# Autodesk Inventor assembly: body
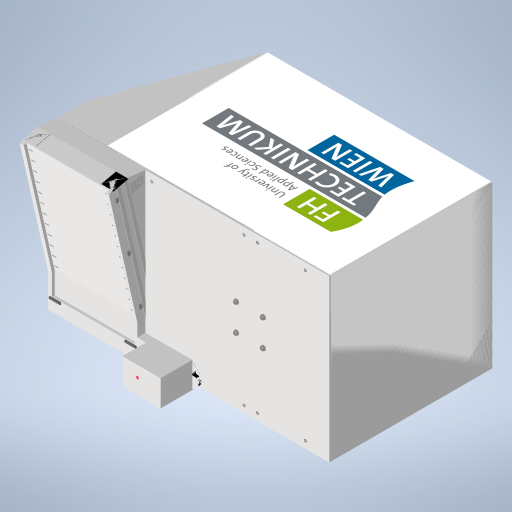
[picture p0: Inventor's stored thumbnail of the model, 512x512]
Saved by Autodesk Inventor 2023 (Build 270158000, 158)
## iProperties
Created: 2023-08-22
Part Number: body
Document SubType Name: Assembly
Designer: chriboehm
Mass: 21023.1 g
Surface Area: 80290.1 cm^2
Volume: 12132.8 cm^3
Density: 1.73275 g/cm^3
Author: chriboehm
## Documents named in this file (28)
- C:\work\robots\butler_2.0\body_model\body.iam
- C:\work\robots\butler_2.0\body_model\parts\Profil 40 x 40 L 450.ipt
- C:\work\robots\butler_2.0\body_model\parts\Profil 40 x 40 L 120.ipt
- C:\work\robots\butler_2.0\body_model\parts\Profil 40 x 40 L 670.ipt
- C:\work\robots\butler_2.0\body_model\parts\Profil 40 x 40 L 540.ipt
- C:\work\robots\butler_2.0\body_model\parts\Profil 40 x 40 L 456.ipt
- C:\work\robots\butler_2.0\body_model\parts\Profil 40 x 40 L 161.ipt
- C:\work\robots\butler_2.0\body_model\parts\Elbow joint 40\Elbow joint 40.iam
- C:\work\robots\butler_2.0\body_model\parts\Reader\RF622A.iam
- C:\work\robots\butler_2.0\body_model\parts\Roller track L 250\Roller track L 250.iam
- C:\work\robots\butler_2.0\body_model\parts\Roller track L 178\Roller track L 178.iam
- C:\work\robots\butler_2.0\body_model\parts\Cap 40_40\Cap 40_40.iam
- C:\work\robots\butler_2.0\body_model\parts\Cap 40_80\Cap 40_80.iam
- C:\work\robots\butler_2.0\body_model\parts\Corner bracket 40_50\Corner bracket 40_50.iam
- C:\work\robots\butler_2.0\body_model\parts\plate_top_01.ipt
- C:\Users\chriboehm\Documents\Inventor\Content Center Files\R2023\en-US\DIN 7984\DIN 7984 - M6 x 12.ipt
- C:\Users\chriboehm\Documents\Inventor\Content Center Files\R2023\en-US\DIN 125-2  A\DIN 125-2 - A 6,4A.ipt
- C:\work\robots\butler_2.0\body_model\parts\plate_top_02.ipt
- C:\work\robots\butler_2.0\body_model\parts\plate_top_03.ipt
- C:\work\robots\butler_2.0\body_model\parts\plate_front.ipt
- C:\work\robots\butler_2.0\body_model\parts\plate_back.ipt
- C:\work\robots\butler_2.0\body_model\parts\plate_side_blank.ipt
- C:\work\robots\butler_2.0\body_model\parts\plate_side_with_logo.ipt
- C:\work\robots\butler_2.0\body_model\parts\emergancy_stop\G_IC03_XX_12648V.iam
- C:\Users\chriboehm\Documents\Inventor\Content Center Files\R2023\en-US\DIN 6912\DIN 6912 - M8 x 20.ipt
- C:\Users\chriboehm\Documents\Inventor\Content Center Files\R2023\en-US\DIN 125-2  A\DIN 125-2 - A 8,4A.ipt
- C:\work\robots\butler_2.0\body_model\body_collision.ipt
- C:\work\robots\butler_2.0\body_model\parts\logo.png
## Components (73 placed, 26 different names)
1. Profil 40 x 40 L 450:1 — Mate:28, Flush:49, Flush:50, Flush:52, Mate:30, Mate:31, Mate:38, Flush:65, Mate:39, Flush:67, Mate:42, Flush:68, Flush:77
2. Profil 40 x 40 L 450:2 — Mate:24, Flush:43, Flush:44, Mate:26, Flush:47, Mate:31, Mate:40, Flush:66, Mate:41, Mate:43, Flush:69, Flush:70, Flush:75
3. Profil 40 x 40 L 120:1 — Mate:33, Flush:55, Flush:56, Mate:34, Flush:57, Flush:58, Angle:2, Angle:3
4. Profil 40 x 40 L 670:1 — Mate:1, Flush:1, Flush:2, Mate:2, Flush:3, Flush:4
5. Profil 40 x 40 L 670:2 — Mate:13, Mate:14, Flush:25, Flush:26, Flush:27, Flush:28, Mate:18, Flush:33, Mate:20, Flush:35, Mate:29, Flush:51, Flush:80, Flush:81, Tangent:2
6. Profil 40 x 40 L 670:3 — Mate:15, Mate:16, Flush:29, Flush:30, Flush:31, Flush:32, Mate:17, Flush:34, Mate:19, Flush:36, Mate:27, Flush:48, Mate:48, Flush:78
7. Profil 40 x 40 L 670:4 — Mate:7, Mate:8, Flush:13, Flush:14, Flush:15, Flush:16
8. Profil 40 x 40 L 540:1 — Mate:5, Flush:9, Flush:10, Mate:8, Flush:13, Flush:14, Mate:10, Flush:17, Flush:18, Mate:13, Flush:27, Flush:28, Mate:22, Flush:39, Flush:40, Flush:79, Mate:99, Mate:104, Mate:113
9. Profil 40 x 40 L 540:2 — Mate:6, Flush:11, Flush:12, Mate:7, Flush:15, Flush:16, Mate:12, Flush:21, Flush:22, Mate:14, Flush:25, Flush:26
10. Profil 40 x 40 L 540:3 — Mate:2, Flush:3, Flush:4, Mate:4, Flush:7, Flush:8, Mate:9, Flush:19, Flush:20, Flush:29, Mate:21, Flush:37, Flush:38
11. Profil 40 x 40 L 540:4 — Mate:1, Flush:1, Flush:2, Mate:3, Flush:5, Flush:6, Mate:11, Flush:23, Flush:24, Mate:15, Flush:31, Mate:97, Flush:85, Mate:101
12. Profil 40 x 40 L 456:1 — Mate:3, Flush:5, Flush:6, Mate:6, Flush:11, Flush:12
13. Profil 40 x 40 L 456:2 — Mate:4, Flush:7, Flush:8, Mate:5, Flush:9, Flush:10
14. Profil 40 x 40 L 456:3 — Mate:11, Mate:12, Flush:21, Flush:22, Flush:23, Flush:24, Flush:32, Mate:46, Mate:78, Flush:82
15. Profil 40 x 40 L 456:4 — Mate:9, Mate:10, Flush:17, Flush:18, Flush:19, Flush:20, Mate:16, Flush:30, Mate:50
16. Profil 40 x 40 L 456:5 — Mate:19, Mate:20, Flush:35, Flush:36, Mate:47, Mate:60
17. Profil 40 x 40 L 456:6 — Mate:17, Mate:18, Flush:33, Flush:34, Mate:46, Mate:47, Tangent:1
18. Profil 40 x 40 L 161:1 — Mate:22, Flush:39, Flush:40, Mate:25, Flush:45, Flush:46, Mate:32, Flush:53, Flush:54, Angle:2, Mate:44, Flush:71, Flush:72
19. Profil 40 x 40 L 161:2 — Mate:21, Flush:37, Flush:38, Mate:23, Flush:41, Flush:42, Mate:45, Flush:73, Flush:74, Mate:49, Flush:76
20. Elbow joint 40:1 [sub-assembly] — Mate:25, Flush:45, Flush:46, Mate:26, Flush:47
21. Elbow joint 40:2 [sub-assembly] — Mate:23, Flush:41, Flush:42, Mate:24, Flush:43, Flush:44
22. Elbow joint 40:3 [sub-assembly] — Mate:27, Flush:48, Mate:28, Flush:49, Flush:50
23. Elbow joint 40:4 [sub-assembly] — Mate:29, Flush:51, Flush:52, Mate:30, Mate:51, Mate:61
24. Elbow joint 40:5 [sub-assembly] — Mate:32, Flush:53, Flush:54, Mate:33, Flush:55, Flush:56
25. Elbow joint 40:6 [sub-assembly] — Mate:34, Flush:57, Flush:58, Mate:95, Flush:83, Flush:84
26. RF622A:1 [sub-assembly] — Mate:95, Flush:83, Flush:84, Angle:3
27. Roller track L 250:1 [sub-assembly] — Mate:37, Flush:63, Flush:64, Mate:40, Flush:66, Mate:41
28. Roller track L 250:2 [sub-assembly] — Flush:61, Flush:62, Mate:36, Mate:38
29. Roller track L 178:1 [sub-assembly] — Mate:37, Flush:63, Flush:64
30. Roller track L 178:2 [sub-assembly] — Flush:61, Flush:62, Mate:36, Flush:65, Mate:39
31. Cap 40_40:1 [sub-assembly] — Mate:45, Flush:73, Flush:74
32. Cap 40_40:4 [sub-assembly] — Mate:44, Flush:71, Flush:72
33. Cap 40_80:1 [sub-assembly] — Mate:43, Flush:69, Flush:70
34. Cap 40_80:2 [sub-assembly] — Flush:67, Mate:42, Flush:68
35. Corner bracket 40_50:1 [sub-assembly] — Mate:48, Flush:77, Flush:78
36. Corner bracket 40_50:2 [sub-assembly] — Mate:49, Flush:75, Flush:76
37. plate_top_01:1 — Mate:50, Flush:79, Mate:51, Mate:56, Mate:57, Mate:58, Mate:59, Mate:100
38. DIN 7984 M6 x 12:1 — Mate:52, Mate:53, Mate:56
39. DIN 7984 M6 x 12:2 — Mate:54, Mate:55, Mate:57
40. DIN 125-2 A A 6,4:1 — Mate:52, Mate:53, Mate:59
41. DIN 125-2 A A 6,4:2 — Mate:54, Mate:55, Mate:58
42. plate_top_02:1 — Mate:60, Mate:61, Flush:80, Mate:70, Mate:71, Mate:72, Mate:73, Mate:74, Mate:75, Mate:76, Mate:102, Mate:105, Mate:107, Mate:108
43. DIN 7984 M6 x 12:3 — Mate:72
44. DIN 125-2 A A 6,4:3 — Mate:73
45. DIN 7984 M6 x 12:4 — Mate:70
46. DIN 125-2 A A 6,4:4 — Mate:71
47. DIN 7984 M6 x 12:5 — Mate:76
48. DIN 125-2 A A 6,4:5 — Mate:109
49. DIN 7984 M6 x 12:6 — Mate:74
50. DIN 125-2 A A 6,4:6 — Mate:75
51. plate_top_03:1 — Mate:78, Flush:81, Flush:82, Mate:87, Mate:88, Mate:89, Mate:90, Mate:91, Mate:92, Mate:93, Mate:94, Mate:98, Mate:122, Mate:123, Mate:124
52. DIN 7984 M6 x 12:7 — Mate:91
53. DIN 125-2 A A 6,4:7 — Mate:92
54. DIN 7984 M6 x 12:8 — Mate:93
55. DIN 125-2 A A 6,4:8 — Mate:94
56. DIN 7984 M6 x 12:9 — Mate:89
57. DIN 125-2 A A 6,4:9 — Mate:90
58. DIN 7984 M6 x 12:10 — Mate:87
59. DIN 125-2 A A 6,4:10 — Mate:88
60. plate_front:1 — Mate:97, Mate:98, Flush:85, Mate:111, Mate:112, Flush:86, Flush:87
61. plate_back:1 — Mate:99, Mate:100, Mate:103, Mate:106, Mate:113
62. plate_side_blank:1 — Mate:101, Mate:102, Mate:103, Angle:4, Mate:110
63. plate_side_with_logo:1 — Mate:104, Mate:105, Mate:106
64. G_IC03_XX_12648V:1 [sub-assembly] — Mate:107, Mate:108, Angle:4, Mate:109
65. body_collision:1 — Flush:86, Flush:87
66. DIN 6912 M8 x 20:1 — Mate:114, Mate:115, Tangent:1, Tangent:2
67. DIN 125-2 A A 8,4:1 — Mate:114, Mate:115, Mate:124
68. DIN 6912 M8 x 20:2
69. DIN 125-2 A A 8,4:2
70. DIN 6912 M8 x 20:3
71. DIN 125-2 A A 8,4:3
72. DIN 6912 M8 x 20:4
73. DIN 125-2 A A 8,4:4
## Component patterns: (4 elements, first: DIN 6912 M8 x 20:1 + DIN 125-2 A A 8,4:1)
## Relationships (205: Mate 115, Flush 85, Angle 3, Tangent 2)
- Mate:1: Profil 40 x 40 L 670:1 ↔ Profil 40 x 40 L 540:4
- Flush:1: Profil 40 x 40 L 670:1 ↔ Profil 40 x 40 L 540:4
- Flush:2: Profil 40 x 40 L 670:1 ↔ Profil 40 x 40 L 540:4
- Mate:2: Profil 40 x 40 L 670:1 ↔ Profil 40 x 40 L 540:3
- Flush:3: Profil 40 x 40 L 670:1 ↔ Profil 40 x 40 L 540:3
- Flush:4: Profil 40 x 40 L 670:1 ↔ Profil 40 x 40 L 540:3
- Mate:3: Profil 40 x 40 L 540:4 ↔ Profil 40 x 40 L 456:1
- Flush:5: Profil 40 x 40 L 540:4 ↔ Profil 40 x 40 L 456:1
- Flush:6: Profil 40 x 40 L 540:4 ↔ Profil 40 x 40 L 456:1
- Mate:4: Profil 40 x 40 L 540:3 ↔ Profil 40 x 40 L 456:2
- Flush:7: Profil 40 x 40 L 540:3 ↔ Profil 40 x 40 L 456:2
- Flush:8: Profil 40 x 40 L 540:3 ↔ Profil 40 x 40 L 456:2
- Mate:5: Profil 40 x 40 L 540:1 ↔ Profil 40 x 40 L 456:2
- Flush:9: Profil 40 x 40 L 540:1 ↔ Profil 40 x 40 L 456:2
- Flush:10: Profil 40 x 40 L 540:1 ↔ Profil 40 x 40 L 456:2
- Mate:6: Profil 40 x 40 L 540:2 ↔ Profil 40 x 40 L 456:1
- Flush:11: Profil 40 x 40 L 540:2 ↔ Profil 40 x 40 L 456:1
- Flush:12: Profil 40 x 40 L 540:2 ↔ Profil 40 x 40 L 456:1
- Mate:7: Profil 40 x 40 L 670:4 ↔ Profil 40 x 40 L 540:2
- Mate:8: Profil 40 x 40 L 670:4 ↔ Profil 40 x 40 L 540:1
- Flush:13: Profil 40 x 40 L 670:4 ↔ Profil 40 x 40 L 540:1
- Flush:14: Profil 40 x 40 L 670:4 ↔ Profil 40 x 40 L 540:1
- Flush:15: Profil 40 x 40 L 670:4 ↔ Profil 40 x 40 L 540:2
- Flush:16: Profil 40 x 40 L 670:4 ↔ Profil 40 x 40 L 540:2
- Mate:9: Profil 40 x 40 L 540:3 ↔ Profil 40 x 40 L 456:4
- Mate:10: Profil 40 x 40 L 540:1 ↔ Profil 40 x 40 L 456:4
- Flush:17: Profil 40 x 40 L 540:1 ↔ Profil 40 x 40 L 456:4
- Flush:18: Profil 40 x 40 L 540:1 ↔ Profil 40 x 40 L 456:4
- Flush:19: Profil 40 x 40 L 540:3 ↔ Profil 40 x 40 L 456:4
- Flush:20: Profil 40 x 40 L 540:3 ↔ Profil 40 x 40 L 456:4
- Mate:11: Profil 40 x 40 L 540:4 ↔ Profil 40 x 40 L 456:3
- Mate:12: Profil 40 x 40 L 540:2 ↔ Profil 40 x 40 L 456:3
- Flush:21: Profil 40 x 40 L 540:2 ↔ Profil 40 x 40 L 456:3
- Flush:22: Profil 40 x 40 L 540:2 ↔ Profil 40 x 40 L 456:3
- Flush:23: Profil 40 x 40 L 540:4 ↔ Profil 40 x 40 L 456:3
- Flush:24: Profil 40 x 40 L 540:4 ↔ Profil 40 x 40 L 456:3
- Mate:13: Profil 40 x 40 L 670:2 ↔ Profil 40 x 40 L 540:1
- Mate:14: Profil 40 x 40 L 670:2 ↔ Profil 40 x 40 L 540:2
- Flush:25: Profil 40 x 40 L 670:2 ↔ Profil 40 x 40 L 540:2
- Flush:26: Profil 40 x 40 L 670:2 ↔ Profil 40 x 40 L 540:2
- Flush:27: Profil 40 x 40 L 670:2 ↔ Profil 40 x 40 L 540:1
- Flush:28: Profil 40 x 40 L 670:2 ↔ Profil 40 x 40 L 540:1
- Mate:15: Profil 40 x 40 L 670:3 ↔ Profil 40 x 40 L 540:4
- Mate:16: Profil 40 x 40 L 670:3 ↔ Profil 40 x 40 L 456:4
- Flush:29: Profil 40 x 40 L 670:3 ↔ Profil 40 x 40 L 540:3
- Flush:30: Profil 40 x 40 L 670:3 ↔ Profil 40 x 40 L 456:4
- Flush:31: Profil 40 x 40 L 670:3 ↔ Profil 40 x 40 L 540:4
- Flush:32: Profil 40 x 40 L 670:3 ↔ Profil 40 x 40 L 456:3
- Mate:17: Profil 40 x 40 L 670:3 ↔ Profil 40 x 40 L 456:6
- Mate:18: Profil 40 x 40 L 670:2 ↔ Profil 40 x 40 L 456:6
- Flush:33: Profil 40 x 40 L 670:2 ↔ Profil 40 x 40 L 456:6
- Flush:34: Profil 40 x 40 L 670:3 ↔ Profil 40 x 40 L 456:6
- Mate:19: Profil 40 x 40 L 670:3 ↔ Profil 40 x 40 L 456:5
- Mate:20: Profil 40 x 40 L 670:2 ↔ Profil 40 x 40 L 456:5
- Flush:35: Profil 40 x 40 L 670:2 ↔ Profil 40 x 40 L 456:5
- Flush:36: Profil 40 x 40 L 670:3 ↔ Profil 40 x 40 L 456:5
- Mate:21: Profil 40 x 40 L 540:3 ↔ Profil 40 x 40 L 161:2
- Flush:37: Profil 40 x 40 L 540:3 ↔ Profil 40 x 40 L 161:2
- Flush:38: Profil 40 x 40 L 540:3 ↔ Profil 40 x 40 L 161:2
- Mate:22: Profil 40 x 40 L 540:1 ↔ Profil 40 x 40 L 161:1
- Flush:39: Profil 40 x 40 L 540:1 ↔ Profil 40 x 40 L 161:1
- Flush:40: Profil 40 x 40 L 540:1 ↔ Profil 40 x 40 L 161:1
- Mate:23: Profil 40 x 40 L 161:2 ↔ Elbow joint 40:2
- Flush:41: Profil 40 x 40 L 161:2 ↔ Elbow joint 40:2
- Flush:42: Profil 40 x 40 L 161:2 ↔ Elbow joint 40:2
- Mate:24: Profil 40 x 40 L 450:2 ↔ Elbow joint 40:2
- Flush:43: Profil 40 x 40 L 450:2 ↔ Elbow joint 40:2
- Flush:44: Profil 40 x 40 L 450:2 ↔ Elbow joint 40:2
- Mate:25: Profil 40 x 40 L 161:1 ↔ Elbow joint 40:1
- Flush:45: Profil 40 x 40 L 161:1 ↔ Elbow joint 40:1
- Flush:46: Profil 40 x 40 L 161:1 ↔ Elbow joint 40:1
- Mate:26: Profil 40 x 40 L 450:2 ↔ Elbow joint 40:1
- Flush:47: Profil 40 x 40 L 450:2 ↔ Elbow joint 40:1
- Mate:27: Profil 40 x 40 L 670:3 ↔ Elbow joint 40:3
- Flush:48: Profil 40 x 40 L 670:3 ↔ Elbow joint 40:3
- Mate:28: Profil 40 x 40 L 450:1 ↔ Elbow joint 40:3
- Flush:49: Profil 40 x 40 L 450:1 ↔ Elbow joint 40:3
- Flush:50: Profil 40 x 40 L 450:1 ↔ Elbow joint 40:3
- Mate:29: Profil 40 x 40 L 670:2 ↔ Elbow joint 40:4
- Flush:51: Profil 40 x 40 L 670:2 ↔ Elbow joint 40:4
- Flush:52: Profil 40 x 40 L 450:1 ↔ Elbow joint 40:4
- Mate:30: Profil 40 x 40 L 450:1 ↔ Elbow joint 40:4
- Mate:31 (217 mm): Profil 40 x 40 L 450:1 ↔ Profil 40 x 40 L 450:2
- Mate:32: Profil 40 x 40 L 161:1 ↔ Elbow joint 40:5
- Flush:53: Profil 40 x 40 L 161:1 ↔ Elbow joint 40:5
- Flush:54 (70 mm): Profil 40 x 40 L 161:1 ↔ Elbow joint 40:5
- Mate:33: Profil 40 x 40 L 120:1 ↔ Elbow joint 40:5
- Flush:55: Profil 40 x 40 L 120:1 ↔ Elbow joint 40:5
- Flush:56: Profil 40 x 40 L 120:1 ↔ Elbow joint 40:5
- Mate:34: Profil 40 x 40 L 120:1 ↔ Elbow joint 40:6
- Flush:57: Profil 40 x 40 L 120:1 ↔ Elbow joint 40:6
- Flush:58: Profil 40 x 40 L 120:1 ↔ Elbow joint 40:6
- Angle:2 (75 deg): Profil 40 x 40 L 120:1 ↔ Profil 40 x 40 L 161:1
- Flush:61: Roller track L 250:2 ↔ Roller track L 178:2
- Flush:62: Roller track L 250:2 ↔ Roller track L 178:2
- Mate:36: Roller track L 250:2 ↔ Roller track L 178:2
- Mate:37: Roller track L 250:1 ↔ Roller track L 178:1
- Flush:63: Roller track L 250:1 ↔ Roller track L 178:1
- Flush:64: Roller track L 250:1 ↔ Roller track L 178:1
- Mate:38: Profil 40 x 40 L 450:1 ↔ Roller track L 250:2
- Flush:65: Profil 40 x 40 L 450:1 ↔ Roller track L 178:2
- Mate:39: Profil 40 x 40 L 450:1 ↔ Roller track L 178:2
- Mate:40: Profil 40 x 40 L 450:2 ↔ Roller track L 250:1
- Flush:66: Profil 40 x 40 L 450:2 ↔ Roller track L 250:1
- Mate:41: Profil 40 x 40 L 450:2 ↔ Roller track L 250:1
- Flush:67: Profil 40 x 40 L 450:1 ↔ Cap 40_80:2
- Mate:42: Profil 40 x 40 L 450:1 ↔ Cap 40_80:2
- Flush:68: Profil 40 x 40 L 450:1 ↔ Cap 40_80:2
- Mate:43: Profil 40 x 40 L 450:2 ↔ Cap 40_80:1
- Flush:69: Profil 40 x 40 L 450:2 ↔ Cap 40_80:1
- Flush:70: Profil 40 x 40 L 450:2 ↔ Cap 40_80:1
- Mate:44: Profil 40 x 40 L 161:1 ↔ Cap 40_40:4
- Mate:45: Profil 40 x 40 L 161:2 ↔ Cap 40_40:1
- Flush:71: Profil 40 x 40 L 161:1 ↔ Cap 40_40:4
- Flush:72: Profil 40 x 40 L 161:1 ↔ Cap 40_40:4
- Flush:73: Profil 40 x 40 L 161:2 ↔ Cap 40_40:1
- Flush:74: Profil 40 x 40 L 161:2 ↔ Cap 40_40:1
- Mate:46 (155 mm): Profil 40 x 40 L 456:3 ↔ Profil 40 x 40 L 456:6
- Mate:47 (50 mm): Profil 40 x 40 L 456:5 ↔ Profil 40 x 40 L 456:6
- Mate:48: Profil 40 x 40 L 670:3 ↔ Corner bracket 40_50:1
- Mate:49: Profil 40 x 40 L 161:2 ↔ Corner bracket 40_50:2
- Flush:75: Profil 40 x 40 L 450:2 ↔ Corner bracket 40_50:2
- Flush:76: Profil 40 x 40 L 161:2 ↔ Corner bracket 40_50:2
- Flush:77: Profil 40 x 40 L 450:1 ↔ Corner bracket 40_50:1
- Flush:78: Profil 40 x 40 L 670:3 ↔ Corner bracket 40_50:1
- Mate:50: Profil 40 x 40 L 456:4 ↔ plate_top_01:1
- Flush:79 (-3 mm): Profil 40 x 40 L 540:1 ↔ plate_top_01:1
- Mate:51 (1 mm): Elbow joint 40:4 ↔ plate_top_01:1
- Mate:52: DIN 7984 M6 x 12:1 ↔ DIN 125-2 A A 6,4:1
- Mate:53: DIN 7984 M6 x 12:1 ↔ DIN 125-2 A A 6,4:1
- Mate:54: DIN 7984 M6 x 12:2 ↔ DIN 125-2 A A 6,4:2
- Mate:55: DIN 7984 M6 x 12:2 ↔ DIN 125-2 A A 6,4:2
- Mate:56: plate_top_01:1 ↔ DIN 7984 M6 x 12:1
- Mate:57: plate_top_01:1 ↔ DIN 7984 M6 x 12:2
- Mate:58: plate_top_01:1 ↔ DIN 125-2 A A 6,4:2
- Mate:59: plate_top_01:1 ↔ DIN 125-2 A A 6,4:1
- Mate:60: Profil 40 x 40 L 456:5 ↔ plate_top_02:1
- Mate:61 (1 mm): Elbow joint 40:4 ↔ plate_top_02:1
- Flush:80 (3 mm): Profil 40 x 40 L 670:2 ↔ plate_top_02:1
- [Mate]: DIN 7984 M6 x 12:3 ↔ DIN 125-2 A A 6,4:3
- [Mate]: DIN 7984 M6 x 12:3 ↔ DIN 125-2 A A 6,4:3
- [Mate]: DIN 7984 M6 x 12:4 ↔ DIN 125-2 A A 6,4:4
- [Mate]: DIN 7984 M6 x 12:4 ↔ DIN 125-2 A A 6,4:4
- [Mate]: DIN 7984 M6 x 12:5 ↔ DIN 125-2 A A 6,4:5
- [Mate]: DIN 7984 M6 x 12:5 ↔ DIN 125-2 A A 6,4:5
- [Mate]: DIN 7984 M6 x 12:6 ↔ DIN 125-2 A A 6,4:6
- [Mate]: DIN 7984 M6 x 12:6 ↔ DIN 125-2 A A 6,4:6
- Mate:70: plate_top_02:1 ↔ DIN 7984 M6 x 12:4
- Mate:71: plate_top_02:1 ↔ DIN 125-2 A A 6,4:4
- Mate:72: plate_top_02:1 ↔ DIN 7984 M6 x 12:3
- Mate:73: plate_top_02:1 ↔ DIN 125-2 A A 6,4:3
- Mate:74: plate_top_02:1 ↔ DIN 7984 M6 x 12:6
- Mate:75: plate_top_02:1 ↔ DIN 125-2 A A 6,4:6
- Mate:76: plate_top_02:1 ↔ DIN 7984 M6 x 12:5
- Mate:78: Profil 40 x 40 L 456:3 ↔ plate_top_03:1
- Flush:81 (-3 mm): Profil 40 x 40 L 670:2 ↔ plate_top_03:1
- Flush:82 (-3 mm): Profil 40 x 40 L 456:3 ↔ plate_top_03:1
- [Mate]: DIN 7984 M6 x 12:7 ↔ DIN 125-2 A A 6,4:7
- [Mate]: DIN 7984 M6 x 12:7 ↔ DIN 125-2 A A 6,4:7
- [Mate]: DIN 7984 M6 x 12:8 ↔ DIN 125-2 A A 6,4:8
- [Mate]: DIN 7984 M6 x 12:8 ↔ DIN 125-2 A A 6,4:8
- [Mate]: DIN 7984 M6 x 12:9 ↔ DIN 125-2 A A 6,4:9
- [Mate]: DIN 7984 M6 x 12:9 ↔ DIN 125-2 A A 6,4:9
- [Mate]: DIN 7984 M6 x 12:10 ↔ DIN 125-2 A A 6,4:10
- [Mate]: DIN 7984 M6 x 12:10 ↔ DIN 125-2 A A 6,4:10
- Mate:87: plate_top_03:1 ↔ DIN 7984 M6 x 12:10
- Mate:88: plate_top_03:1 ↔ DIN 125-2 A A 6,4:10
- Mate:89: plate_top_03:1 ↔ DIN 7984 M6 x 12:9
- Mate:90: plate_top_03:1 ↔ DIN 125-2 A A 6,4:9
- Mate:91: plate_top_03:1 ↔ DIN 7984 M6 x 12:7
- Mate:92: plate_top_03:1 ↔ DIN 125-2 A A 6,4:7
- Mate:93: plate_top_03:1 ↔ DIN 7984 M6 x 12:8
- Mate:94: plate_top_03:1 ↔ DIN 125-2 A A 6,4:8
- Mate:95: Elbow joint 40:6 ↔ RF622A:1
- Flush:83 (-2.5 mm): Elbow joint 40:6 ↔ RF622A:1
- Flush:84 (-2.5 mm): Elbow joint 40:6 ↔ RF622A:1
- Angle:3 (-90 deg): Profil 40 x 40 L 120:1 ↔ RF622A:1
- Mate:97: Profil 40 x 40 L 540:4 ↔ plate_front:1
- Mate:98: plate_top_03:1 ↔ plate_front:1
- Flush:85 (-3 mm): Profil 40 x 40 L 540:4 ↔ plate_front:1
- Mate:99: Profil 40 x 40 L 540:1 ↔ plate_back:1
- Mate:100: plate_top_01:1 ↔ plate_back:1
- Mate:101: Profil 40 x 40 L 540:4 ↔ plate_side_blank:1
- Mate:102: plate_top_02:1 ↔ plate_side_blank:1
- Mate:103: plate_back:1 ↔ plate_side_blank:1
- Mate:104: Profil 40 x 40 L 540:1 ↔ plate_side_with_logo:1
- Mate:105: plate_top_02:1 ↔ plate_side_with_logo:1
- Mate:106: plate_back:1 ↔ plate_side_with_logo:1
- Mate:107: plate_top_02:1 ↔ G_IC03_XX_12648V:1
- Mate:108: plate_top_02:1 ↔ G_IC03_XX_12648V:1
- Angle:4 (0 deg): plate_side_blank:1 ↔ G_IC03_XX_12648V:1
- Mate:109: DIN 125-2 A A 6,4:5 ↔ G_IC03_XX_12648V:1
- Mate:110: plate_side_blank:1
- Mate:111: plate_front:1
- Mate:112: plate_front:1
- Mate:113: Profil 40 x 40 L 540:1 ↔ plate_back:1
- Mate:114: DIN 6912 M8 x 20:1 ↔ DIN 125-2 A A 8,4:1
- Mate:115: DIN 6912 M8 x 20:1 ↔ DIN 125-2 A A 8,4:1
- Mate:122: plate_top_03:1
- Mate:123: plate_top_03:1
- Mate:124 (8 mm): plate_top_03:1 ↔ DIN 125-2 A A 8,4:1
- Tangent:1 (3 mm): Profil 40 x 40 L 456:6 ↔ DIN 6912 M8 x 20:1
- Tangent:2 (-227 mm): Profil 40 x 40 L 670:2 ↔ DIN 6912 M8 x 20:1
- Flush:86: plate_front:1 ↔ body_collision:1
- Flush:87: plate_front:1 ↔ body_collision:1
## Named parameters: d146_d135 = 0 mm, d147_d136 = 0 mm, d148_d135 = 0 mm, d149_d136 = 0 mm, d150_d135 = 0 mm, d151_d136 = 0 mm, d152_d135 = 0 mm, d153_d136 = 0 mm, d165_d146_d135 = 0 mm, d166_d147_d136 = 0 mm, d167_d146_d135 = 0 mm, d168_d147_d136 = 0 mm, d169_d146_d135 = 0 mm, d170_d147_d136 = 0 mm, d171_d146_d135 = 0 mm, d172_d147_d136 = 0 mm
